# Autodesk Inventor assembly: Case
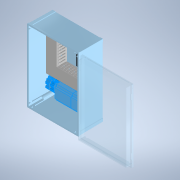
[picture p0: Inventor's stored thumbnail of the model, 180x180]
Saved by Autodesk Inventor 2020 (Build 240168000, 168)
## iProperties
Created: 2019-12-11
Part Number: Case
Document SubType Name: Assembly
Designer: nicoc
Author: nicoc
## Documents named in this file (7)
- D:\Repos\P5-AIonFPGA\cad\Case\Case.iam
- D:\Repos\P5-AIonFPGA\cad\Case\FIBOX_Bottom.ipt
- D:\Repos\P5-AIonFPGA\cad\Case\FIBOX_Top.ipt
- D:\Repos\P5-AIonFPGA\cad\Case\Ultra96\PWB_USDEV1-1_FINAL.iam
- D:\Repos\P5-AIonFPGA\cad\Case\Terminalblock\Terminalblock.iam
- D:\Repos\P5-AIonFPGA\cad\Case\SlottedWiring\SlottexWiring200mm.ipt
- D:\Repos\P5-AIonFPGA\cad\Case\SlottedWiring\SlottexWiring110mm.ipt
## Components (7 placed, 6 different names)
1. FIBOX_Bottom:1 — Mate:1, Mate:2, Mate:3, Mate:4, Mate:5, Mate:7
2. FIBOX_Top:1 — Mate:1
3. PWB_USDEV1-1_FINAL:1 [sub-assembly] — Mate:2
4. Terminalblock:1 [sub-assembly] — Mate:3, Mate:9
5. SlottexWiring200mm:1 — Mate:4, Mate:8, Flush:2
6. SlottexWiring200mm:2 — Mate:5, Mate:6, Flush:1, Mate:9
7. SlottexWiring110mm:1 — Mate:6, Flush:1, Mate:7, Mate:8, Flush:2
## Relationships (11: Mate 9, Flush 2)
- Mate:1: FIBOX_Bottom:1 ↔ FIBOX_Top:1
- Mate:2: FIBOX_Bottom:1 ↔ PWB_USDEV1-1_FINAL:1
- Mate:3: FIBOX_Bottom:1 ↔ Terminalblock:1
- Mate:4: FIBOX_Bottom:1 ↔ SlottexWiring200mm:1
- Mate:5: FIBOX_Bottom:1 ↔ SlottexWiring200mm:2
- Mate:6: SlottexWiring200mm:2 ↔ SlottexWiring110mm:1
- Flush:1: SlottexWiring200mm:2 ↔ SlottexWiring110mm:1
- Mate:7: FIBOX_Bottom:1 ↔ SlottexWiring110mm:1
- Mate:8: SlottexWiring200mm:1 ↔ SlottexWiring110mm:1
- Flush:2: SlottexWiring200mm:1 ↔ SlottexWiring110mm:1
- Mate:9 (5 mm): Terminalblock:1 ↔ SlottexWiring200mm:2
